# Autodesk Inventor assembly: CL3-200
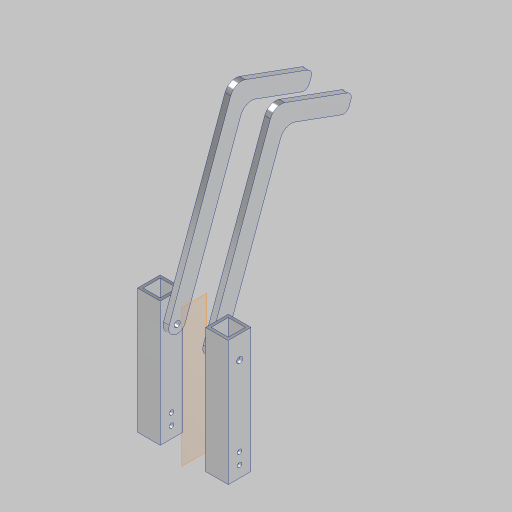
[picture p0: Inventor's stored thumbnail of the model, 512x512]
Saved by Autodesk Inventor 2023.5 (Build 275446000, 446)
## iProperties
Created: 2025-01-30
Part Number: CL3-200
Document SubType Name: Assembly
Designer: slick
Author: slick
## Documents named in this file (3)
- C:\Users\slick\OneDrive\Desktop\2025-ReefScape---CAD\Climber\CHD1\CL3-200.iam
- C:\Users\slick\OneDrive\Desktop\2025-ReefScape---CAD\Climber\CHD1\CHD-003.ipt
- C:\Users\slick\OneDrive\Desktop\2025-ReefScape---CAD\Climber\CHD1\CHD-002.ipt
## Components (4 placed, 2 different names)
1. CHD-003:1 — Flush:1, Flush:2, Mate:1, Insert:1, Symmetry:1
2. CHD-003:2 — Flush:1, Flush:2, Mate:1, Insert:2, Symmetry:1
3. CHD-002:1 — Insert:1, Flush:3
4. CHD-002:2 — Insert:2, Flush:3
## Relationships (7: Flush 3, Insert 2, Mate 1, Symmetry 1)
- Flush:1: CHD-003:1 ↔ CHD-003:2
- Flush:2: CHD-003:1 ↔ CHD-003:2
- Mate:1 (50.8 mm): CHD-003:1 ↔ CHD-003:2
- Insert:1: CHD-003:1 ↔ CHD-002:1
- Insert:2: CHD-003:2 ↔ CHD-002:2
- Flush:3: CHD-002:1 ↔ CHD-002:2
- Symmetry:1: CHD-003:1 ↔ CHD-003:2
